# Autodesk Inventor assembly: Wilwood Dynalite 4 Piston Caliper 120-5082
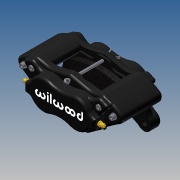
[picture p0: Inventor's stored thumbnail of the model, 180x180]
Saved by Autodesk Inventor 2012 SP1 (Build 160190100, 190)
## iProperties
Created: 2012-02-18
Part Number: Wilwood Dynalite 4 Piston Caliper 120-5082
Project: Alphan
Document SubType Name: Assembly
Designer: A.COMEAU
Author: A.COMEAU
## Documents named in this file (7)
- C:\Users\Comeau\Dropbox\Projet Alpha\R&D\3D_MODEL\PURCHASED PARTS\Willwood\Caliper dynalite\Wilwood Dynalite 4 Piston Caliper 120-5082.iam
- C:\Users\Comeau\Dropbox\Projet Alpha\R&D\3D_MODEL\PURCHASED PARTS\Willwood\Caliper dynalite\BRAKE PAD.ipt
- C:\Users\Comeau\Dropbox\Projet Alpha\R&D\3D_MODEL\PURCHASED PARTS\Willwood\Caliper dynalite\Wilwood Dynalite 4 Piston Caliper .81 inch Rotor Thickness.ipt
- C:\Users\Comeau\Dropbox\Projet Alpha\R&D\3D_MODEL\PURCHASED PARTS\QUINCAILLERIE\fr-FR\ANSI B18.3(05)\ANSI B18.3 - 10-24 UNC - 0,5(31).ipt
- C:\Users\Comeau\Dropbox\Projet Alpha\R&D\3D_MODEL\PURCHASED PARTS\QUINCAILLERIE\fr-FR\ISO 7089\ISO 7089 - 5 - 140 HV(1).ipt
- C:\Users\Comeau\Dropbox\Projet Alpha\R&D\3D_MODEL\PURCHASED PARTS\QUINCAILLERIE\fr-FR\JIS B 1575  A\JIS B 1575 - M 6 x 1 F.ipt
- C:\Users\Comeau\Dropbox\Projet Alpha\R&D\3D_MODEL\PURCHASED PARTS\QUINCAILLERIE\fr-FR\SAE J487a\SAE J487a - 5_32 x 3   Type fourche.ipt
## Components (14 placed, 6 different names)
1. Wilwood Dynalite 4 Piston Caliper .81 inch Rotor Thickness:1 — Placage:1, Placage:2, Placage:3, Affleurement:1, Placage:4, Placage:8, Placage:9, Placage:10, Placage:11, Placage:12, Logement:1, Logement:2, Logement:3, Logement:4, Logement:5, Logement:6, Placage:20, Placage:21
2. BRAKE PAD:2 — Placage:1, Placage:6, Placage:7, Placage:8
3. BRAKE PAD:3 — Placage:2, Placage:6, Placage:7
4. ISO 7089 5 - 140 HV:2 — Placage:9, Placage:10, Placage:18
5. ISO 7089 5 - 140 HV:1 — Placage:11, Placage:12, Placage:19
6. Vis cylindrique à six pans creux - Pouce N° 10 - 24 UNC - 1/2:2 — Placage:18
7. Vis cylindrique à six pans creux - Pouce N° 10 - 24 UNC - 1/2:1 — Placage:19
8. Vis cylindrique à six pans creux - Pouce N° 10 - 24 UNC - 1/2:3 — Logement:2
9. Vis cylindrique à six pans creux - Pouce N° 10 - 24 UNC - 1/2:4 — Logement:1
10. JIS B 1575 A - Métrique M 6 F:1 — Logement:5
11. JIS B 1575 A - Métrique M 6 F:2 — Logement:4
12. JIS B 1575 A - Métrique M 6 F:3 — Logement:6
13. JIS B 1575 A - Métrique M 6 F:4 — Logement:3
14. Goupille - Clavette - Type fourche (Pouce) SAE J487a 5/32 x 3   Type fourche:1 — Placage:20, Placage:21
## Relationships (24: Mate 17, Insert 6, Flush 1)
- Placage:1 [Mate]: Wilwood Dynalite 4 Piston Caliper .81 inch Rotor Thickness:1 ↔ BRAKE PAD:2
- Placage:2 [Mate]: Wilwood Dynalite 4 Piston Caliper .81 inch Rotor Thickness:1 ↔ BRAKE PAD:3
- Placage:3 [Mate] (24.892 mm): Wilwood Dynalite 4 Piston Caliper .81 inch Rotor Thickness:1
- Affleurement:1 [Flush]: Wilwood Dynalite 4 Piston Caliper .81 inch Rotor Thickness:1
- Placage:4 [Mate]: Wilwood Dynalite 4 Piston Caliper .81 inch Rotor Thickness:1
- Placage:6 [Mate]: BRAKE PAD:2 ↔ BRAKE PAD:3
- Placage:7 [Mate]: BRAKE PAD:2 ↔ BRAKE PAD:3
- Placage:8 [Mate]: Wilwood Dynalite 4 Piston Caliper .81 inch Rotor Thickness:1 ↔ BRAKE PAD:2
- Placage:10 [Mate]: Wilwood Dynalite 4 Piston Caliper .81 inch Rotor Thickness:1 ↔ ISO 7089 5 - 140 HV:2
- Placage:12 [Mate]: Wilwood Dynalite 4 Piston Caliper .81 inch Rotor Thickness:1 ↔ ISO 7089 5 - 140 HV:1
- Placage:18 [Mate]: ISO 7089 5 - 140 HV:2 ↔ Vis cylindrique à six pans creux - Pouce N° 10 - 24 UNC - 1/2:2
- Placage:19 [Mate]: ISO 7089 5 - 140 HV:1 ↔ Vis cylindrique à six pans creux - Pouce N° 10 - 24 UNC - 1/2:1
- Logement:1 [Insert]: Wilwood Dynalite 4 Piston Caliper .81 inch Rotor Thickness:1 ↔ Vis cylindrique à six pans creux - Pouce N° 10 - 24 UNC - 1/2:4
- Logement:2 [Insert]: Wilwood Dynalite 4 Piston Caliper .81 inch Rotor Thickness:1 ↔ Vis cylindrique à six pans creux - Pouce N° 10 - 24 UNC - 1/2:3
- Logement:3 [Insert]: Wilwood Dynalite 4 Piston Caliper .81 inch Rotor Thickness:1 ↔ JIS B 1575 A - Métrique M 6 F:4
- Logement:4 [Insert]: Wilwood Dynalite 4 Piston Caliper .81 inch Rotor Thickness:1 ↔ JIS B 1575 A - Métrique M 6 F:2
- Logement:5 [Insert]: Wilwood Dynalite 4 Piston Caliper .81 inch Rotor Thickness:1 ↔ JIS B 1575 A - Métrique M 6 F:1
- Logement:6 [Insert]: Wilwood Dynalite 4 Piston Caliper .81 inch Rotor Thickness:1 ↔ JIS B 1575 A - Métrique M 6 F:3
- Placage:20 [Mate]: Wilwood Dynalite 4 Piston Caliper .81 inch Rotor Thickness:1 ↔ Goupille - Clavette - Type fourche (Pouce) SAE J487a 5/32 x 3   Type fourche:1
- Placage:21 [Mate]: Wilwood Dynalite 4 Piston Caliper .81 inch Rotor Thickness:1 ↔ Goupille - Clavette - Type fourche (Pouce) SAE J487a 5/32 x 3   Type fourche:1
- Placage:9 [Mate]: Wilwood Dynalite 4 Piston Caliper .81 inch Rotor Thickness:1 ↔ ISO 7089 5 - 140 HV:2
- Placage:11 [Mate]: Wilwood Dynalite 4 Piston Caliper .81 inch Rotor Thickness:1 ↔ ISO 7089 5 - 140 HV:1
- [Mate]: Wilwood Dynalite 4 Piston Caliper .81 inch Rotor Thickness:1 ↔ Vis cylindrique à six pans creux - Pouce N° 10 - 24 UNC - 1/2:2
- [Mate]: Wilwood Dynalite 4 Piston Caliper .81 inch Rotor Thickness:1 ↔ Vis cylindrique à six pans creux - Pouce N° 10 - 24 UNC - 1/2:1
